# Autodesk Inventor assembly: ASY GBK 3210 wall shield Center 3
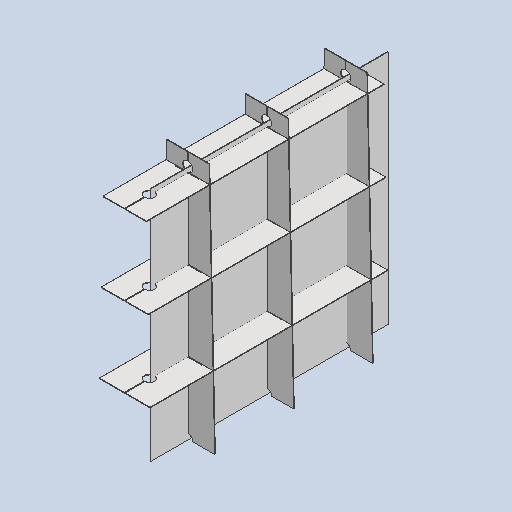
[picture p0: Inventor's stored thumbnail of the model, 512x512]
Saved by Autodesk Inventor 2026 (Build 300175000, 175)
## iProperties
Created: 2026-05-19
Part Number: ASY GBK 3210 wall shield Center 3
Document SubType Name: Assembly
Designer: pokla
Mass: 152628 g
Surface Area: 99280.6 cm^2
Volume: 19443.1 cm^3
Density: 7.85 g/cm^3
Author: admin
## Documents named in this file (6)
- C:\Users\pokla\Documents\Inventor\GBK-Gubkinskiy\ASY GBK 3210 wall shield Center 3.iam
- C:\Users\pokla\Documents\Inventor\GBK-Gubkinskiy\GBK 3201 Center second rib.ipt
- C:\Users\pokla\Documents\Inventor\GBK-Gubkinskiy\GBK 3202 stringer 4.ipt
- C:\Users\pokla\Documents\Inventor\GBK-Gubkinskiy\GBK 3203 stringer 5.ipt
- C:\Users\pokla\Documents\Inventor\GBK-Gubkinskiy\GBK 3204 stringer 6.ipt
- C:\Users\pokla\Documents\Inventor\GBK-Gubkinskiy\010.7 GBK shield.ipt
## Components (13 placed, 5 different names)
1. 0713 GBK stringer C1.ipt:1 — Жесткий:1
2. 0714 GBK stringer C2.ipt:1 — Жесткий:2
3. 0715 GBK stringer C3.ipt:1 — Жесткий:3
4. 0713 GBK stringer C1.ipt:2 — Жесткий:6
5. 0714 GBK stringer C2.ipt:2 — Жесткий:5
6. 0715 GBK stringer C3.ipt:2 — Жесткий:4
7. 010.7 GBK shield.ipt:1 — Совмещение:7, Совмещение:8
8. 0711 GBK Center rib 2.ipt:1 — Заподлицо:4, Жесткий:1, Жесткий:2, Жесткий:3, Совмещение:6
9. 0711 GBK Center rib 2.ipt:2 — Заподлицо:4, Совмещение:5, Жесткий:4, Жесткий:5, Жесткий:6
10. 0711 GBK Center rib 2.ipt:3
11. 0711 GBK Center rib 2.ipt:4
12. 0711 GBK Center rib 2.ipt:5
13. 0711 GBK Center rib 2.ipt:6
## Component patterns: (3 elements, first: 0711 GBK Center rib 2.ipt:1 + 0711 GBK Center rib 2.ipt:2)
## Relationships (11: WeldJoint 6, Mate 4, Flush 1)
- Заподлицо:4 [Flush]: 0711 GBK Center rib 2.ipt:1 ↔ 0711 GBK Center rib 2.ipt:2
- Жесткий:1 [WeldJoint] (4 mm): 0713 GBK stringer C1.ipt:1 ↔ 0711 GBK Center rib 2.ipt:1
- Жесткий:2 [WeldJoint] (4 mm): 0714 GBK stringer C2.ipt:1 ↔ 0711 GBK Center rib 2.ipt:1
- Жесткий:3 [WeldJoint] (4 mm): 0715 GBK stringer C3.ipt:1 ↔ 0711 GBK Center rib 2.ipt:1
- Совмещение:5 [Mate]: 0711 GBK Center rib 2.ipt:2
- Совмещение:6 [Mate]: 0711 GBK Center rib 2.ipt:1
- Жесткий:4 [WeldJoint] (4 mm): 0715 GBK stringer C3.ipt:2 ↔ 0711 GBK Center rib 2.ipt:2
- Жесткий:5 [WeldJoint] (4 mm): 0714 GBK stringer C2.ipt:2 ↔ 0711 GBK Center rib 2.ipt:2
- Жесткий:6 [WeldJoint] (4 mm): 0713 GBK stringer C1.ipt:2 ↔ 0711 GBK Center rib 2.ipt:2
- Совмещение:7 [Mate]: 010.7 GBK shield.ipt:1
- Совмещение:8 [Mate]: 010.7 GBK shield.ipt:1
